# Autodesk Inventor assembly: solenoid assy
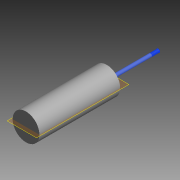
[picture p0: Inventor's stored thumbnail of the model, 180x180]
Saved by Autodesk Inventor 2015 (Build 190159000, 159)
## iProperties
Created: 2015-09-23
Part Number: solenoid assy
Document SubType Name: Assembly
Designer: francis
Author: francis
## Documents named in this file (3)
- C:\Users\francis\Documents\GitHub\CAD\solenoid assy.iam
- C:\Users\francis\Documents\GitHub\CAD\solenoid_body.ipt
- C:\Users\francis\Documents\GitHub\CAD\shaft.ipt
## Components (2 placed, 2 different names)
1. solenoid_body:1 — Cylindrical:1
2. shaft:1 — Cylindrical:1
## Relationships (1: CylindricalJoint 1)
- Cylindrical:1: solenoid_body:1 ↔ shaft:1
